# Autodesk Inventor assembly: Modul
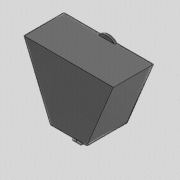
[picture p0: Inventor's stored thumbnail of the model, 180x180]
Saved by Autodesk Inventor 2018 (Build 220112000, 112)
## iProperties
Company: Fraunhofer ILT
Created: 2018-10-15
Part Number: Modul
Material: geeigneten Werkstoff auswählen !
Document SubType Name: Assembly
Designer: N.Grubert
Title: =Description
Author: N.Grubert
## Documents named in this file (5)
- C:\Users\knabe\Documents\GitHub\COSIMA-Laserstar\CAD\Detektormodul\Detektormodul.iam
- C:\Users\knabe\Documents\GitHub\COSIMA-Laserstar\CAD\Oktagongehäuse\Detektormodul Deckel.ipt
- C:\Users\knabe\Documents\GitHub\COSIMA-Laserstar\CAD\Oktagongehäuse\Detektormodul Gehäuse.ipt
- C:\Users\knabe\Documents\GitHub\COSIMA-Laserstar\CAD\Detektormodul\DetektorElektronik_Stage1.iam
- C:\Users\knabe\Documents\GitHub\COSIMA-Laserstar\CAD\Detektormodul\DetektorElektronik_Stage2.iam
## Components (4 placed, 4 different names)
1. Detektormodul Deckel:1 — Passend:1, Fluchtend:10, Fluchtend:11
2. Detektormodul Gehäuse:1 — Passend:1, Passend:2, Passend:3, Passend:4, Passend:5, Passend:6, Fluchtend:10, Fluchtend:11, Passend:19, Passend:20, Passend:21, Passend:22
3. DetektorElektronik_Stage1:1 [sub-assembly] — Passend:5, Passend:6, Passend:22
4. DetektorElektronik_Stage2:1 [sub-assembly] — Passend:19, Passend:20, Passend:21
## Relationships (12: Mate 10, Flush 2)
- Passend:1 [Mate]: Detektormodul Deckel:1 ↔ Detektormodul Gehäuse:1
- Passend:2 [Mate]: Detektormodul Gehäuse:1
- Passend:3 [Mate]: Detektormodul Gehäuse:1
- Passend:4 [Mate]: Detektormodul Gehäuse:1
- Passend:5 [Mate]: Detektormodul Gehäuse:1 ↔ DetektorElektronik_Stage1:1
- Passend:6 [Mate] (0.5 mm): Detektormodul Gehäuse:1 ↔ DetektorElektronik_Stage1:1
- Fluchtend:10 [Flush]: Detektormodul Deckel:1 ↔ Detektormodul Gehäuse:1
- Fluchtend:11 [Flush]: Detektormodul Deckel:1 ↔ Detektormodul Gehäuse:1
- Passend:19 [Mate] (0.5 mm): Detektormodul Gehäuse:1 ↔ DetektorElektronik_Stage2:1
- Passend:20 [Mate]: Detektormodul Gehäuse:1 ↔ DetektorElektronik_Stage2:1
- Passend:21 [Mate] (0.5 mm): Detektormodul Gehäuse:1 ↔ DetektorElektronik_Stage2:1
- Passend:22 [Mate] (1 mm): Detektormodul Gehäuse:1 ↔ DetektorElektronik_Stage1:1
